# Autodesk Inventor assembly: Assembly
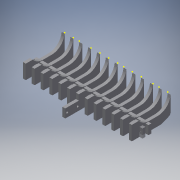
[picture p0: Inventor's stored thumbnail of the model, 180x180]
Saved by Autodesk Inventor 2017 (Build 210142000, 142)
## iProperties
Created: 2017-05-10
Part Number: Assembly
Document SubType Name: Assembly
Designer: s4461999
Author: s4461999
## Documents named in this file (7)
- U:\CAD\SecondClaw\Design\Assembly.iam
- U:\CAD\SecondClaw\Design\brace.ipt
- U:\CAD\SecondClaw\Design\CenterFinger.ipt
- U:\CAD\SecondClaw\Design\Finger.ipt
- U:\CAD\SecondClaw\Design\Finger_MIR.ipt
- U:\CAD\SecondClaw\Design\Finger_MIR1.ipt
- U:\CAD\SecondClaw\Design\Finger_MIR1_MIR.ipt
## Components (15 placed, 6 different names)
1. brace:1 — Rigid:2
2. brace:2 — Rigid:1, Rigid:4, Rigid:5, Rigid:6, Rigid:7, Rigid:8
3. CenterFinger:1 — Rigid:1, Rigid:2, Flush:1
4. Finger:1 — Rigid:4, Flush:2
5. Finger:3 — Rigid:6
6. Finger:4 — Rigid:5
7. Finger:5 — Rigid:8
8. Finger:9 — Rigid:7
9. Finger_MIR:1
10. Finger_MIR:2
11. Finger_MIR:3
12. Finger_MIR:4
13. Finger_MIR:5
14. Finger_MIR1:1
15. Finger_MIR1_MIR:1
## Relationships (9: WeldJoint 7, Flush 2)
- Rigid:1 [WeldJoint]: brace:2 ↔ CenterFinger:1
- Rigid:2 [WeldJoint]: brace:1 ↔ CenterFinger:1
- Rigid:4 [WeldJoint]: brace:2 ↔ Finger:1
- Rigid:5 [WeldJoint]: brace:2 ↔ Finger:4
- Rigid:6 [WeldJoint]: brace:2 ↔ Finger:3
- Rigid:7 [WeldJoint]: brace:2 ↔ Finger:9
- Rigid:8 [WeldJoint]: brace:2 ↔ Finger:5
- Flush:1 (-2.5 mm): CenterFinger:1
- Flush:2 (-2.5 mm): Finger:1
